# Autodesk Inventor assembly: MonteCarloM1.2
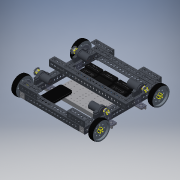
[picture p0: Inventor's stored thumbnail of the model, 180x180]
Saved by Autodesk Inventor 2016 (Build 200138000, 138)
## iProperties
Created: 2015-09-05
Part Number: MonteCarloM1.2
Document SubType Name: Assembly
Designer: Tim
Author: Tim
## Documents named in this file (12)
- C:\Users\Tim\Documents\GitHub\phi_robotics\3d-models\FTC_Tetrix_KOP_Block_Party\Tim Bloot Designs\MonteCarloM1.2.iam
- C:\Users\Tim\Documents\GitHub\phi_robotics\3d-models\FTC_Tetrix_KOP_Block_Party\Tim Bloot Designs\MonteCarloM1.1.iam
- C:\Users\Tim\Documents\GitHub\phi_robotics\3d-models\FTC_Tetrix_KOP_Block_Party\Tetrix_Kit_FTC\Autodesk Inventor Files\tetrix_motor_mount-old.ipt
- C:\Users\Tim\Documents\GitHub\phi_robotics\3d-models\FTC_Tetrix_KOP_Block_Party\Tetrix_Kit_FTC\Autodesk Inventor Files\tetrix_motor.iam
- C:\Users\Tim\Documents\GitHub\phi_robotics\3d-models\FTC_Tetrix_KOP_Block_Party\Tetrix_Kit_FTC\Autodesk Inventor Files\tetrix_c_channel-5.ipt
- C:\Users\Tim\Documents\GitHub\phi_robotics\3d-models\FTC_Tetrix_KOP_Block_Party\Tetrix_Kit_FTC\Autodesk Inventor Files\tetrix_c_channel-round.ipt
- C:\Users\Tim\Documents\GitHub\phi_robotics\3d-models\FTC_Tetrix_KOP_Block_Party\Tim Bloot Designs\MCPlate2.ipt
- C:\Users\Tim\Documents\GitHub\phi_robotics\3d-models\FTC_Tetrix_KOP_Block_Party\Tim Bloot Designs\SmallCGearN'MLock.iam
- C:\Users\Tim\Documents\GitHub\phi_robotics\3d-models\FTC_Tetrix_KOP_Block_Party\Tetrix_Kit_FTC\Autodesk Inventor Files\tetrix_motor_controller.ipt
- C:\Users\Tim\Documents\GitHub\phi_robotics\3d-models\FTC_Tetrix_KOP_Block_Party\Tetrix_Kit_FTC\Autodesk Inventor Files\tetrix_servo_controller.ipt
- C:\Users\Tim\Documents\GitHub\phi_robotics\3d-models\FTC_Tetrix_KOP_Block_Party\Tim Bloot Designs\Andoid Phone.ipt
- C:\Users\Tim\Documents\GitHub\phi_robotics\3d-models\FTC_Tetrix_KOP_Block_Party\Tim Bloot Designs\Phone Mount.ipt
## Components (22 placed, 11 different names)
1. MonteCarloM1.1:1 [sub-assembly] — Rigid:1, Rigid:2, Rigid:3, Rigid:4, Rigid:7, Rigid:8, Rigid:9, Rigid:10
2. tetrix_motor_mount-old:1 — Rigid:3, Rotational:1
3. tetrix_motor_mount-old:2 — Rigid:1, Rotational:3
4. tetrix_motor_mount-old:3 — Rigid:2, Rotational:4
5. tetrix_motor_mount-old:4 — Rigid:4, Rotational:2
6. tetrix_motor:1 [sub-assembly] — Rotational:1, Rigid:12
7. tetrix_motor:2 [sub-assembly] — Rotational:2, Rigid:11
8. tetrix_motor:4 [sub-assembly] — Rotational:4, Rigid:14
9. tetrix_motor:5 [sub-assembly] — Rotational:3, Rigid:13
10. tetrix_c_channel-5:1
11. tetrix_c_channel-round:1 — Rigid:7
12. tetrix_c_channel-round:2 — Rigid:8
13. MCPlate2:1 — Rigid:9, Rigid:10, Rigid:15, Rigid:16, Rigid:18
14. SmallCGearN'MLock:1 [sub-assembly] — Rigid:13
15. SmallCGearN'MLock:2 [sub-assembly] — Rigid:14
16. SmallCGearN'MLock:3 [sub-assembly] — Rigid:12
17. SmallCGearN'MLock:4 [sub-assembly] — Rigid:11
18. tetrix_motor_controller:1 — Rigid:15
19. tetrix_motor_controller:2 — Rigid:16, Rigid:17
20. tetrix_servo_controller:1 — Rigid:17
21. Phone Mount:1 — Rigid:18, Mate:1
22. Andoid Phone:1 — Mate:1
## Relationships (23: WeldJoint 18, RevoluteJoint 4, Mate 1)
- Rigid:1 [WeldJoint]: MonteCarloM1.1:1 ↔ tetrix_motor_mount-old:2
- Rigid:2 [WeldJoint]: MonteCarloM1.1:1 ↔ tetrix_motor_mount-old:3
- Rigid:3 [WeldJoint]: MonteCarloM1.1:1 ↔ tetrix_motor_mount-old:1
- Rigid:4 [WeldJoint]: MonteCarloM1.1:1 ↔ tetrix_motor_mount-old:4
- Rotational:1 [RevoluteJoint]: tetrix_motor_mount-old:1 ↔ tetrix_motor:1
- Rotational:2 [RevoluteJoint]: tetrix_motor_mount-old:4 ↔ tetrix_motor:2
- Rotational:3 [RevoluteJoint]: tetrix_motor_mount-old:2 ↔ tetrix_motor:5
- Rotational:4 [RevoluteJoint]: tetrix_motor_mount-old:3 ↔ tetrix_motor:4
- [WeldJoint]: tetrix_c_channel-5:1 ↔ tetrix_c_channel-round:1
- [WeldJoint]: tetrix_c_channel-5:1 ↔ tetrix_c_channel-round:2
- Rigid:7 [WeldJoint] (0.25 mm): MonteCarloM1.1:1 ↔ tetrix_c_channel-round:1
- Rigid:8 [WeldJoint] (0.25 mm): MonteCarloM1.1:1 ↔ tetrix_c_channel-round:2
- Rigid:9 [WeldJoint]: MonteCarloM1.1:1 ↔ MCPlate2:1
- Rigid:10 [WeldJoint]: MonteCarloM1.1:1 ↔ MCPlate2:1
- Rigid:11 [WeldJoint] (-11.5 mm): tetrix_motor:2 ↔ SmallCGearN'MLock:4
- Rigid:12 [WeldJoint] (-11.5 mm): tetrix_motor:1 ↔ SmallCGearN'MLock:3
- Rigid:13 [WeldJoint] (-11.5 mm): tetrix_motor:5 ↔ SmallCGearN'MLock:1
- Rigid:14 [WeldJoint] (-11.5 mm): tetrix_motor:4 ↔ SmallCGearN'MLock:2
- Rigid:15 [WeldJoint]: MCPlate2:1 ↔ tetrix_motor_controller:1
- Rigid:16 [WeldJoint]: MCPlate2:1 ↔ tetrix_motor_controller:2
- Rigid:17 [WeldJoint]: tetrix_motor_controller:2 ↔ tetrix_servo_controller:1
- Rigid:18 [WeldJoint]: MCPlate2:1 ↔ Phone Mount:1
- Mate:1: Phone Mount:1 ↔ Andoid Phone:1
